# Autodesk Inventor assembly: Baterías
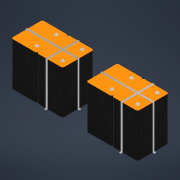
[picture p0: Inventor's stored thumbnail of the model, 180x180]
Saved by Autodesk Inventor 2022 (Build 260153000, 153)
## iProperties
Created: 2021-10-01
Part Number: Baterías
Document SubType Name: Assembly
Designer: seb_0
Mass: 33006.4 g
Surface Area: 8204.7 cm^2
Volume: 18507.6 cm^3
Density: 1.7834 g/cm^3
Author: seb_0
## Documents named in this file (3)
- D:\Documentos\15.PUCP_2021-2\[PDM] Proyecto de Diseño Mecatrónico\ProyectoGIT\ProyectoRobotPallet\Batería\Baterías.iam
- D:\Documentos\15.PUCP_2021-2\[PDM] Proyecto de Diseño Mecatrónico\ProyectoGIT\ProyectoRobotPallet\Batería\Batería.ipt
- D:\Documentos\15.PUCP_2021-2\[PDM] Proyecto de Diseño Mecatrónico\ProyectoGIT\ProyectoRobotPallet\Batería\Soporte.ipt
## Components (6 placed, 2 different names)
1. Batería:1 — Coincidencia:1, Coincidencia:2, Nivelación:1, Coincidencia:3, Nivelación:2, Nivelación:3, Coincidencia:6, Coincidencia:7, Coincidencia:8
2. Batería:2 — Coincidencia:3, Nivelación:2, Nivelación:3, Coincidencia:4, Nivelación:4, Nivelación:5
3. Batería:3 — Coincidencia:4, Nivelación:4, Nivelación:5, Coincidencia:5, Nivelación:6, Nivelación:7, Coincidencia:9
4. Batería:4 — Coincidencia:5, Nivelación:6, Nivelación:7, Coincidencia:10, Coincidencia:11
5. Soporte:1 — Coincidencia:6, Coincidencia:7, Coincidencia:8
6. Soporte:2 — Coincidencia:9, Coincidencia:10, Coincidencia:11
## Relationships (18: Mate 11, Flush 7)
- Coincidencia:1 [Mate]: Batería:1
- Coincidencia:2 [Mate]: Batería:1
- Nivelación:1 [Flush]: Batería:1
- Coincidencia:3 [Mate]: Batería:1 ↔ Batería:2
- Nivelación:2 [Flush]: Batería:1 ↔ Batería:2
- Nivelación:3 [Flush]: Batería:1 ↔ Batería:2
- Coincidencia:4 [Mate] (150 mm): Batería:2 ↔ Batería:3
- Nivelación:4 [Flush]: Batería:2 ↔ Batería:3
- Nivelación:5 [Flush]: Batería:2 ↔ Batería:3
- Coincidencia:5 [Mate]: Batería:3 ↔ Batería:4
- Nivelación:6 [Flush]: Batería:3 ↔ Batería:4
- Nivelación:7 [Flush]: Batería:3 ↔ Batería:4
- Coincidencia:6 [Mate]: Batería:1 ↔ Soporte:1
- Coincidencia:7 [Mate]: Batería:1 ↔ Soporte:1
- Coincidencia:8 [Mate]: Batería:1 ↔ Soporte:1
- Coincidencia:9 [Mate]: Batería:3 ↔ Soporte:2
- Coincidencia:10 [Mate]: Batería:4 ↔ Soporte:2
- Coincidencia:11 [Mate]: Batería:4 ↔ Soporte:2
